# Autodesk Inventor assembly: CamComplete
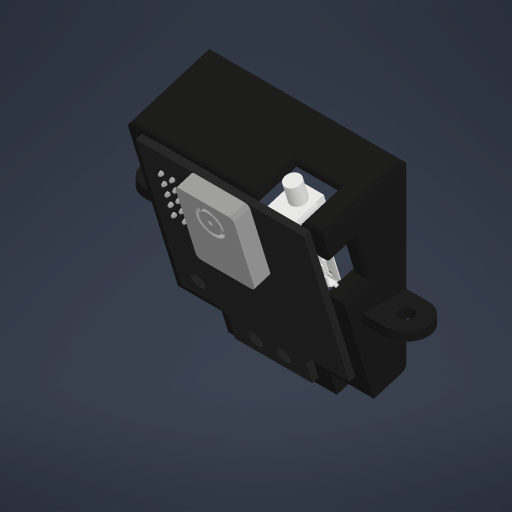
[picture p0: Inventor's stored thumbnail of the model, 512x512]
Saved by Autodesk Inventor 2023 (Build 270158000, 158)
## iProperties
Created: 2023-05-12
Part Number: CamComplete
Document SubType Name: Assembly
Designer: Elias Braun
Author: Elias Braun
## Documents named in this file (3)
- C:\Users\Elias Braun\Nextcloud2\RoboCup2023\Cam\CamComplete.iam
- C:\Users\Elias Braun\Nextcloud2\RoboCup2023\Cam\Pixy2\pixy2Pixy 2.iam
- C:\Users\Elias Braun\Nextcloud2\RoboCup2023\Cam\Pixy2-Bracket.ipt
## Components (2 placed, 2 different names)
1. Pixy2-Bracket:1 — Mate:1, Mate:2, Mate:3
2. pixy2Pixy 2:1 [sub-assembly] — Mate:1, Mate:2, Mate:3
## Relationships (3: Mate 3)
- Mate:1: Pixy2-Bracket:1 ↔ pixy2Pixy 2:1
- Mate:2: Pixy2-Bracket:1 ↔ pixy2Pixy 2:1
- Mate:3: Pixy2-Bracket:1 ↔ pixy2Pixy 2:1
